# Autodesk Inventor assembly: ASY ДМФ 0100 Барабан v2.0
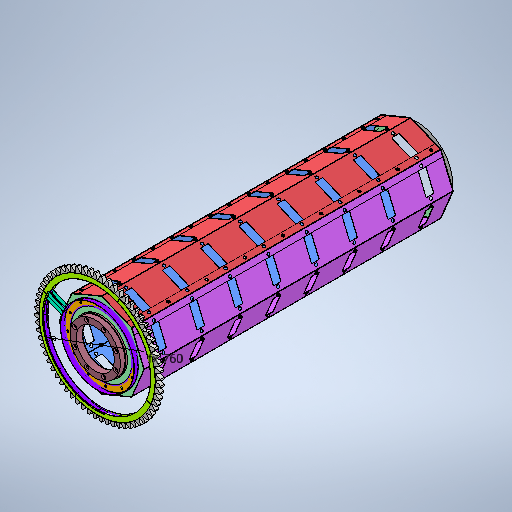
[picture p0: Inventor's stored thumbnail of the model, 512x512]
Saved by Autodesk Inventor 2025 (Build 290162010, 162A)
## iProperties
Created: 2024-04-28
Part Number: ASY ДМФ 0100 Барабан v2.0
Document SubType Name: Assembly
Designer: pokla
Author: pokla
## Documents named in this file (19)
- C:\Users\admin\Yandex.Disk\home pc\Inventor\DMF-Disk-Micro-Filter\ASY ДМФ 0100 Барабан v2.0.iam
- C:\Users\admin\Yandex.Disk\home pc\Inventor\DMF-Disk-Micro-Filter\ДМФ 01 21 Барабан торец НОС v2.0.ipt
- C:\Users\admin\Yandex.Disk\home pc\Inventor\DMF-Disk-Micro-Filter\ДМФ 01 13 Барабан Лист лев брт v2.0.ipt
- C:\Users\admin\Yandex.Disk\home pc\Inventor\DMF-Disk-Micro-Filter\ДМФ 01 14 Барабан Лист прав брт v2.0.ipt
- C:\Users\admin\Yandex.Disk\home pc\Inventor\DMF-Disk-Micro-Filter\ДМФ 01 31 Барабан Опорное кольцо НОС v2.0.ipt
- C:\Users\admin\Yandex.Disk\home pc\Inventor\DMF-Disk-Micro-Filter\ДМФ 01 17 опора крышки v2.0.ipt
- C:\Users\admin\Yandex.Disk\home pc\Inventor\DMF-Disk-Micro-Filter\ДМФ 000 размеры v2.0.ipt
- C:\Users\admin\Yandex.Disk\home pc\Inventor\DMF-Disk-Micro-Filter\ДМФ 01 12 Барабан усилитель v2.0.ipt
- C:\Users\admin\Yandex.Disk\home pc\Inventor\DMF-Disk-Micro-Filter\ASY ДМФ 010 крышка v2.0.iam
- C:\Users\admin\Yandex.Disk\home pc\Inventor\DMF-Disk-Micro-Filter\ДМФ 01 32 Барабан Опорное кольцо КОРМА v2.0.ipt
- C:\Users\admin\Yandex.Disk\home pc\Inventor\DMF-Disk-Micro-Filter\ДМФ 01 22 Барабан торец КОРМА v2.0.ipt
- C:\Users\admin\Yandex.Disk\home pc\Inventor\DMF-Disk-Micro-Filter\ASY фильтр пакет v2.0.iam
- C:\Users\admin\Yandex.Disk\home pc\Inventor\DMF-Disk-Micro-Filter\DMF old version Gleb\ДМФ 01 21 Барабан торец НОС.ipt
- C:\Users\admin\Yandex.Disk\home pc\Inventor\DMF-Disk-Micro-Filter\DMF2.0 01 42 Gear way 2.ipt
- C:\Users\admin\Yandex.Disk\home pc\Inventor\DMF-Disk-Micro-Filter\DMF2.0 01 43 Gear rim 3.ipt
- C:\Users\admin\Yandex.Disk\home pc\Inventor\DMF-Disk-Micro-Filter\DMF2.0 01 44 Gear rim 4.ipt
- C:\Users\admin\Yandex.Disk\home pc\Inventor\DMF-Disk-Micro-Filter\DMF2.0 01 45 Gear ring 5.ipt
- C:\Users\admin\Yandex.Disk\home pc\Inventor\DMF-Disk-Micro-Filter\DMF2.0 01 46 Gear axis wheel 6.ipt
- C:\Users\admin\Yandex.Disk\home pc\Inventor\DMF-Disk-Micro-Filter\Новые шестерни 27.08.2025\sector big gear.ipt
## Components (49 placed, 18 different names)
1. ДМФ 000 размеры v2.0:1 — Rigid:30
2. ДМФ 01 21 Барабан торец НОС v2.0:2 — Mate:15, Flush:8, Flush:9, Flush:10, Flush:11, Mate:16, Mate:17, Mate:19, Mate:21, Flush:15, Flush:16, Flush:17, Mate:23, Rigid:27, Rigid:28, Rigid:29, Rigid:30
3. ДМФ 01 31 Барабан Опорное кольцо НОС v2.0:1 — Rigid:29
4. ДМФ 01 32 Барабан Опорное кольцо КОРМА v2.0:1 — Rigid:20
5. ДМФ 01 22 Барабан торец КОРМА v2.0:1 — Flush:12, Flush:13, Mate:18, Rigid:20
6. ДМФ 01 13 Барабан Лист лев брт v2.0:1 — Flush:10, Flush:11, Mate:16, Flush:13, Mate:18, Mate:20, Mate:29
7. ДМФ 01 14 Барабан Лист прав брт v2.0:1 — Flush:8, Flush:9, Mate:17, Flush:12, Mate:22, Mate:28
8. ДМФ 01 17 опора крышки v2.0:1 — Mate:21, Flush:15, Mate:22
9. ДМФ 01 17 опора крышки v2.0:2 — Mate:19, Mate:20, Mate:27
10. ASY ДМФ 010 крышка v2.0:1 [sub-assembly] — Flush:16, Flush:17, Mate:23, Mate:27
11. ДМФ 01 29 Барабан сборочный лист:1 — Mate:28, Mate:29
12. DMF2.0 01 45 Gear ring 5:1 — Rigid:21, Rigid:22, Rigid:23, Rigid:26, Rigid:27
13. DMF2.0 01 44 Gear rim 4:1 — Rigid:22
14. DMF2.0 01 46 Gear axis wheel 6:1 — Rigid:26
15. ДМФ 01 12 Барабан усилитель v2.0:49 — Mate:30, Tangent:1, Mate:31, Rigid:21, Rigid:25
16. DMF2.0 01 42 Gear way 2:1 — Mate:30, Tangent:1, Mate:31
17. ДМФ 01 12 Барабан усилитель v2.0:50 — Rigid:25
18. ASY фильтр пакет v2.0:1 [sub-assembly] — Mate:24, Mate:25
19. ASY фильтр пакет v2.0:2 [sub-assembly]
20. ASY фильтр пакет v2.0:3 [sub-assembly]
21. ASY фильтр пакет v2.0:4 [sub-assembly]
22. ASY фильтр пакет v2.0:5 [sub-assembly]
23. ASY фильтр пакет v2.0:6 [sub-assembly]
24. ASY фильтр пакет v2.0:7 [sub-assembly]
25. ASY фильтр пакет v2.0:8 [sub-assembly]
26. sector big gear:1 — Rigid:28
27. sector big gear:2
28. sector big gear:3
29. sector big gear:4
30. sector big gear:5
31. sector big gear:6
32. sector big gear:7
33. sector big gear:8
34. sector big gear:9
35. sector big gear:10
36. sector big gear:11
37. sector big gear:12
38. sector big gear:13
39. sector big gear:14
40. sector big gear:15
41. sector big gear:16
42. DMF2.0 01 43 Gear rim 3:2 — Rigid:24
43. DMF2.0 01 43 Gear rim 3:1 — Rigid:23, Rigid:24
44. DMF2.0 01 43 Gear rim 3:3
45. DMF2.0 01 43 Gear rim 3:6
46. DMF2.0 01 43 Gear rim 3:4
47. DMF2.0 01 43 Gear rim 3:7
48. DMF2.0 01 43 Gear rim 3:5
49. DMF2.0 01 43 Gear rim 3:8
## Component patterns: (8 elements, first: ASY фильтр пакет v2.0:1), (16 elements, first: sector big gear:1), (4 elements, first: DMF2.0 01 43 Gear rim 3:2 + DMF2.0 01 43 Gear rim 3:1)
## Relationships (37: Mate 16, WeldJoint 11, Flush 9, Tangent 1)
- Mate:15: ДМФ 01 21 Барабан торец НОС v2.0:2
- Flush:8: ДМФ 01 21 Барабан торец НОС v2.0:2 ↔ ДМФ 01 14 Барабан Лист прав брт v2.0:1
- Flush:9: ДМФ 01 21 Барабан торец НОС v2.0:2 ↔ ДМФ 01 14 Барабан Лист прав брт v2.0:1
- Flush:10: ДМФ 01 21 Барабан торец НОС v2.0:2 ↔ ДМФ 01 13 Барабан Лист лев брт v2.0:1
- Flush:11: ДМФ 01 21 Барабан торец НОС v2.0:2 ↔ ДМФ 01 13 Барабан Лист лев брт v2.0:1
- Mate:16: ДМФ 01 21 Барабан торец НОС v2.0:2 ↔ ДМФ 01 13 Барабан Лист лев брт v2.0:1
- Mate:17: ДМФ 01 21 Барабан торец НОС v2.0:2 ↔ ДМФ 01 14 Барабан Лист прав брт v2.0:1
- Flush:12: ДМФ 01 22 Барабан торец КОРМА v2.0:1 ↔ ДМФ 01 14 Барабан Лист прав брт v2.0:1
- Flush:13: ДМФ 01 22 Барабан торец КОРМА v2.0:1 ↔ ДМФ 01 13 Барабан Лист лев брт v2.0:1
- Mate:18: ДМФ 01 22 Барабан торец КОРМА v2.0:1 ↔ ДМФ 01 13 Барабан Лист лев брт v2.0:1
- Mate:19: ДМФ 01 21 Барабан торец НОС v2.0:2 ↔ ДМФ 01 17 опора крышки v2.0:2
- Mate:20: ДМФ 01 13 Барабан Лист лев брт v2.0:1 ↔ ДМФ 01 17 опора крышки v2.0:2
- Mate:21: ДМФ 01 21 Барабан торец НОС v2.0:2 ↔ ДМФ 01 17 опора крышки v2.0:1
- Flush:15 (-2 mm): ДМФ 01 21 Барабан торец НОС v2.0:2 ↔ ДМФ 01 17 опора крышки v2.0:1
- Mate:22: ДМФ 01 14 Барабан Лист прав брт v2.0:1 ↔ ДМФ 01 17 опора крышки v2.0:1
- Flush:16: ДМФ 01 21 Барабан торец НОС v2.0:2 ↔ ASY ДМФ 010 крышка v2.0:1
- Flush:17: ДМФ 01 21 Барабан торец НОС v2.0:2 ↔ ASY ДМФ 010 крышка v2.0:1
- Mate:23: ДМФ 01 21 Барабан торец НОС v2.0:2 ↔ ASY ДМФ 010 крышка v2.0:1
- Mate:24: ASY фильтр пакет v2.0:1
- Mate:25: ASY фильтр пакет v2.0:1
- Mate:27: ДМФ 01 17 опора крышки v2.0:2 ↔ ASY ДМФ 010 крышка v2.0:1
- Mate:28: ДМФ 01 14 Барабан Лист прав брт v2.0:1 ↔ ДМФ 01 29 Барабан сборочный лист:1
- Mate:29: ДМФ 01 13 Барабан Лист лев брт v2.0:1 ↔ ДМФ 01 29 Барабан сборочный лист:1
- Rigid:20 [WeldJoint]: ДМФ 01 32 Барабан Опорное кольцо КОРМА v2.0:1 ↔ ДМФ 01 22 Барабан торец КОРМА v2.0:1
- Mate:30: ДМФ 01 12 Барабан усилитель v2.0:49 ↔ DMF2.0 01 42 Gear way 2:1
- Tangent:1: ДМФ 01 12 Барабан усилитель v2.0:49 ↔ DMF2.0 01 42 Gear way 2:1
- Mate:31: ДМФ 01 12 Барабан усилитель v2.0:49 ↔ DMF2.0 01 42 Gear way 2:1
- Rigid:21 [WeldJoint]: DMF2.0 01 45 Gear ring 5:1 ↔ ДМФ 01 12 Барабан усилитель v2.0:49
- Rigid:22 [WeldJoint]: DMF2.0 01 45 Gear ring 5:1 ↔ DMF2.0 01 44 Gear rim 4:1
- Rigid:23 [WeldJoint]: DMF2.0 01 45 Gear ring 5:1 ↔ DMF2.0 01 43 Gear rim 3:1
- Rigid:24 [WeldJoint] (25 mm): DMF2.0 01 43 Gear rim 3:2 ↔ DMF2.0 01 43 Gear rim 3:1
- Rigid:25 [WeldJoint] (25 mm): ДМФ 01 12 Барабан усилитель v2.0:49 ↔ ДМФ 01 12 Барабан усилитель v2.0:50
- Rigid:26 [WeldJoint]: DMF2.0 01 45 Gear ring 5:1 ↔ DMF2.0 01 46 Gear axis wheel 6:1
- Rigid:27 [WeldJoint]: ДМФ 01 21 Барабан торец НОС v2.0:2 ↔ DMF2.0 01 45 Gear ring 5:1
- Rigid:28 [WeldJoint]: ДМФ 01 21 Барабан торец НОС v2.0:2 ↔ sector big gear:1
- Rigid:29 [WeldJoint]: ДМФ 01 21 Барабан торец НОС v2.0:2 ↔ ДМФ 01 31 Барабан Опорное кольцо НОС v2.0:1
- Rigid:30 [WeldJoint]: ДМФ 000 размеры v2.0:1 ↔ ДМФ 01 21 Барабан торец НОС v2.0:2
